# Autodesk Inventor assembly: Assembly1
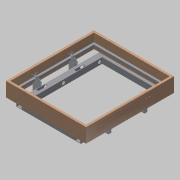
[picture p0: Inventor's stored thumbnail of the model, 180x180]
Saved by Autodesk Inventor 2014 SP1 (Build 180222100, 222)
## iProperties
Created: 2014-01-07
Part Number: Assembly1
Document SubType Name: Assembly
Designer: Rauhul Varma
Author: Rauhul Varma
## Documents named in this file (12)
- C:\Users\Rauhul Varma\Desktop\2014 Base\Assembly1.iam
- C:\Users\Rauhul Varma\Desktop\2014 Base\Tube Mirrored.ipt
- C:\Users\Rauhul Varma\Desktop\2014 Base\Tube.ipt
- C:\Users\Rauhul Varma\Desktop\2014 Base\Back Beam.ipt
- C:\Users\Rauhul Varma\Desktop\2014 Base\Front Beam.ipt
- C:\Users\Rauhul Varma\Desktop\2014 Base\Bumper Rail Stand Top Cap.ipt
- C:\Users\Rauhul Varma\Desktop\2014 Base\Bumper Rail Stand.ipt
- C:\Users\Rauhul Varma\Desktop\2014 Base\Latch.iam
- C:\Users\Rauhul Varma\Desktop\2014 Base\Bumper Rail Side.ipt
- C:\Users\Rauhul Varma\Desktop\2014 Base\Bumper Rail Cross.ipt
- C:\Users\Rauhul Varma\Desktop\2014 Base\Bumper Wood Front.ipt
- C:\Users\Rauhul Varma\Desktop\2014 Base\Bumper Wood Side.ipt
## Components (24 placed, 11 different names)
1. Tube Mirrored:1 — Flush:1, Flush:2, Mate:2, Flush:6, Mate:3, Mate:10, Flush:8, Mate:12, Mate:18, Flush:10, Mate:19, Mate:49
2. Tube:1 — Flush:1, Flush:2, Mate:1, Flush:3, Flush:4, Flush:5, Mate:34, Mate:35, Flush:13, Flush:14, Mate:36, Mate:37
3. Back Beam:1 — Flush:5, Flush:6, Mate:3
4. Front Beam:1 — Mate:1, Flush:3, Flush:4, Mate:2, Flush:17
5. Bumper Rail Stand Top Cap:1 — Mate:6, Mate:7, Flush:7, Mate:8, Mate:9, Mate:11
6. Bumper Rail Stand:1 — Mate:7, Flush:7, Mate:8, Mate:10, Flush:8, Mate:12
7. Latch:1 [sub-assembly] — Mate:6, Mate:9, Mate:11, Mate:50, Mate:51, Mate:52, Mate:53
8. Bumper Rail Stand Top Cap:2
9. Bumper Rail Stand:2 — Mate:18, Flush:10, Mate:19, Mate:20, Mate:21
10. Latch:2 [sub-assembly]
11. Bumper Rail Side:1 — Mate:20, Mate:21, Mate:38, Flush:15, Mate:39, Mate:44
12. Bumper Rail Stand Top Cap:3
13. Bumper Rail Stand:3 — Mate:35, Flush:13, Mate:37
14. Latch:3 [sub-assembly]
15. Bumper Rail Stand Top Cap:4
16. Bumper Rail Stand:4 — Mate:34, Flush:14, Mate:36
17. Latch:4 [sub-assembly]
18. Bumper Rail Side:2 — Mate:40, Flush:16, Mate:41, Mate:42, Mate:43
19. Bumper Rail Cross:1 — Mate:38, Flush:15, Mate:39, Mate:40, Mate:46
20. Bumper Rail Cross:2 — Flush:16, Mate:41, Mate:42, Flush:17, Mate:45
21. Bumper Wood Front:1 — Mate:46, Mate:48, Flush:21, Flush:22
22. Bumper Wood Side:1 — Mate:44, Mate:47, Flush:18, Mate:49, Flush:22, Mate:50, Mate:52, Mate:53
23. Bumper Wood Front:2 — Mate:45, Mate:47, Flush:18, Flush:19, Flush:20
24. Bumper Wood Side:2 — Mate:43, Flush:19, Flush:20, Mate:48, Flush:21
## Relationships (73: Mate 51, Flush 22)
- Flush:1: Tube Mirrored:1 ↔ Tube:1
- Flush:2: Tube Mirrored:1 ↔ Tube:1
- Mate:1: Tube:1 ↔ Front Beam:1
- Flush:3: Tube:1 ↔ Front Beam:1
- Flush:4: Tube:1 ↔ Front Beam:1
- Mate:2: Tube Mirrored:1 ↔ Front Beam:1
- Flush:5: Tube:1 ↔ Back Beam:1
- Flush:6: Tube Mirrored:1 ↔ Back Beam:1
- Mate:3: Tube Mirrored:1 ↔ Back Beam:1
- Mate:6: Bumper Rail Stand Top Cap:1 ↔ Latch:1
- Mate:7: Bumper Rail Stand Top Cap:1 ↔ Bumper Rail Stand:1
- Flush:7: Bumper Rail Stand Top Cap:1 ↔ Bumper Rail Stand:1
- Mate:8: Bumper Rail Stand Top Cap:1 ↔ Bumper Rail Stand:1
- Mate:9: Bumper Rail Stand Top Cap:1 ↔ Latch:1
- Mate:10: Tube Mirrored:1 ↔ Bumper Rail Stand:1
- Flush:8: Tube Mirrored:1 ↔ Bumper Rail Stand:1
- Mate:11: Bumper Rail Stand Top Cap:1 ↔ Latch:1
- Mate:12 (25.4 mm): Tube Mirrored:1 ↔ Bumper Rail Stand:1
- [Mate]: Bumper Rail Stand Top Cap:2 ↔ Latch:2
- [Mate]: Bumper Rail Stand Top Cap:2 ↔ Bumper Rail Stand:2
- [Flush]: Bumper Rail Stand Top Cap:2 ↔ Bumper Rail Stand:2
- [Mate]: Bumper Rail Stand Top Cap:2 ↔ Bumper Rail Stand:2
- [Mate]: Bumper Rail Stand Top Cap:2 ↔ Latch:2
- [Mate]: Bumper Rail Stand Top Cap:2 ↔ Latch:2
- Mate:18: Tube Mirrored:1 ↔ Bumper Rail Stand:2
- Flush:10: Tube Mirrored:1 ↔ Bumper Rail Stand:2
- Mate:19 (25.4 mm): Tube Mirrored:1 ↔ Bumper Rail Stand:2
- Mate:20: Bumper Rail Stand:2 ↔ Bumper Rail Side:1
- Mate:21: Bumper Rail Stand:2 ↔ Bumper Rail Side:1
- [Mate]: Bumper Rail Stand Top Cap:3 ↔ Latch:3
- [Mate]: Bumper Rail Stand Top Cap:3 ↔ Bumper Rail Stand:3
- [Flush]: Bumper Rail Stand Top Cap:3 ↔ Bumper Rail Stand:3
- [Mate]: Bumper Rail Stand Top Cap:3 ↔ Bumper Rail Stand:3
- [Mate]: Bumper Rail Stand Top Cap:3 ↔ Latch:3
- [Mate]: Bumper Rail Stand Top Cap:3 ↔ Latch:3
- [Mate]: Bumper Rail Stand Top Cap:4 ↔ Latch:4
- [Mate]: Bumper Rail Stand Top Cap:4 ↔ Bumper Rail Stand:4
- [Flush]: Bumper Rail Stand Top Cap:4 ↔ Bumper Rail Stand:4
- [Mate]: Bumper Rail Stand Top Cap:4 ↔ Bumper Rail Stand:4
- [Mate]: Bumper Rail Stand Top Cap:4 ↔ Latch:4
- [Mate]: Bumper Rail Stand Top Cap:4 ↔ Latch:4
- [Mate]: Bumper Rail Stand:4 ↔ Bumper Rail Side:2
- [Mate]: Bumper Rail Stand:4 ↔ Bumper Rail Side:2
- Mate:34: Tube:1 ↔ Bumper Rail Stand:4
- Mate:35: Tube:1 ↔ Bumper Rail Stand:3
- Flush:13: Tube:1 ↔ Bumper Rail Stand:3
- Flush:14: Tube:1 ↔ Bumper Rail Stand:4
- Mate:36 (25.4 mm): Tube:1 ↔ Bumper Rail Stand:4
- Mate:37 (25.4 mm): Tube:1 ↔ Bumper Rail Stand:3
- Mate:38: Bumper Rail Side:1 ↔ Bumper Rail Cross:1
- Flush:15: Bumper Rail Side:1 ↔ Bumper Rail Cross:1
- Mate:39: Bumper Rail Side:1 ↔ Bumper Rail Cross:1
- Mate:40: Bumper Rail Side:2 ↔ Bumper Rail Cross:1
- Flush:16: Bumper Rail Side:2 ↔ Bumper Rail Cross:2
- Mate:41: Bumper Rail Side:2 ↔ Bumper Rail Cross:2
- Mate:42: Bumper Rail Side:2 ↔ Bumper Rail Cross:2
- Flush:17 (3.175 mm): Front Beam:1 ↔ Bumper Rail Cross:2
- Mate:43: Bumper Rail Side:2 ↔ Bumper Wood Side:2
- Mate:44: Bumper Rail Side:1 ↔ Bumper Wood Side:1
- Mate:45: Bumper Rail Cross:2 ↔ Bumper Wood Front:2
- Mate:46: Bumper Rail Cross:1 ↔ Bumper Wood Front:1
- Mate:47: Bumper Wood Side:1 ↔ Bumper Wood Front:2
- Flush:18: Bumper Wood Side:1 ↔ Bumper Wood Front:2
- Flush:19: Bumper Wood Front:2 ↔ Bumper Wood Side:2
- Flush:20: Bumper Wood Front:2 ↔ Bumper Wood Side:2
- Mate:48: Bumper Wood Front:1 ↔ Bumper Wood Side:2
- Flush:21: Bumper Wood Front:1 ↔ Bumper Wood Side:2
- Mate:49 (22.225 mm): Tube Mirrored:1 ↔ Bumper Wood Side:1
- Flush:22: Bumper Wood Front:1 ↔ Bumper Wood Side:1
- Mate:50: Latch:1 ↔ Bumper Wood Side:1
- Mate:51: Latch:1
- Mate:52: Latch:1 ↔ Bumper Wood Side:1
- Mate:53: Latch:1 ↔ Bumper Wood Side:1
## Named parameters: d30_d21 = 0 mm, d31_d22 = 0 mm, d32_d23 = 0 mm, d33_d24 = 0 mm, d34_d25 = 0 mm, d35_d28 = 0 mm, d41_d21 = 0 mm, d42_d22 = 0 mm, d43_d23 = 0 mm, d44_d24 = 0 mm, d45_d25 = 0 mm, d46_d28 = 0 mm, d47_d30_d21 = 0 mm, d48_d31_d22 = 0 mm, d49_d32_d23 = 0 mm, d50_d33_d24 = 0 mm, d51_d34_d25 = 0 mm, d52_d35_d28 = 0 mm, d53_d39 = 0 mm, d54_d40 = 0 mm
